# Autodesk Inventor assembly: Pneumatic Eye Bolt
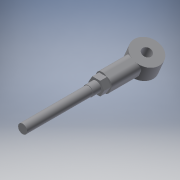
[picture p0: Inventor's stored thumbnail of the model, 180x180]
Saved by Autodesk Inventor 2019.4 (Build 234330000, 330)
## iProperties
Created: 2020-01-29
Part Number: Pneumatic Eye Bolt
Document SubType Name: Assembly
Designer: admin
Author: admin
## Documents named in this file (3)
- C:\Users\admin\Desktop\FRC 2020 Engineering\GitHub\7738-2020\Robot V2\Intake V2\Pneumatic Eye Bolt.iam
- C:\Users\admin\Desktop\FRC 2020 Engineering\GitHub\7738-2020\Robot V2\Intake V2\Eye Bolt.ipt
- C:\Users\admin\Desktop\FRC 2020 Engineering\GitHub\7738-2020\Robot V2\Intake V2\Pneumatic Shaft.ipt
## Components (2 placed, 2 different names)
1. Eye Bolt:1 — Mate:1, Mate:2
2. Pneumatic Shaft:1 — Mate:1, Mate:2
## Relationships (2: Mate 2)
- Mate:1: Eye Bolt:1 ↔ Pneumatic Shaft:1
- Mate:2: Eye Bolt:1 ↔ Pneumatic Shaft:1
